# Autodesk Inventor assembly: Roller
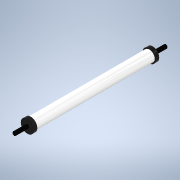
[picture p0: Inventor's stored thumbnail of the model, 180x180]
Saved by Autodesk Inventor 2020 (Build 240168000, 168)
## iProperties
Created: 2020-01-26
Part Number: Roller
Document SubType Name: Assembly
Designer: autum
Author: autum
## Documents named in this file (4)
- C:\Users\autum\Google Drive\Iron Riders 4180 (Roosevelt Robotics)\2019-2020\Build_Design\Robot 2020 (new)\Intake 2.0\Roller.iam
- C:\Users\autum\Google Drive\Iron Riders 4180 (Roosevelt Robotics)\2019-2020\Build_Design\Robot 2020 (new)\Intake 2.0\PVC Roller.ipt
- C:\Users\autum\Google Drive\Iron Riders 4180 (Roosevelt Robotics)\2019-2020\Build_Design\Robot 2020 (new)\Intake 2.0\Hex Adapter.ipt
- C:\Users\autum\Google Drive\Iron Riders 4180 (Roosevelt Robotics)\2019-2020\Build_Design\Robot 2020 (new)\Intake 2.0\Hex Instert.ipt
## Components (5 placed, 3 different names)
1. PVC Roller:1 — Insert:1, Insert:2
2. Hex Adapter:1 — Insert:1, Mate:3, Flush:2, Mate:4
3. Hex Adapter:2 — Insert:2, Mate:1, Mate:2, Flush:1
4. Hex Instert:1 — Mate:3, Flush:2, Mate:4
5. Hex Instert:2 — Mate:1, Mate:2, Flush:1
## Relationships (8: Mate 4, Insert 2, Flush 2)
- Insert:1: PVC Roller:1 ↔ Hex Adapter:1
- Insert:2: PVC Roller:1 ↔ Hex Adapter:2
- Mate:1: Hex Adapter:2 ↔ Hex Instert:2
- Mate:2: Hex Adapter:2 ↔ Hex Instert:2
- Flush:1: Hex Adapter:2 ↔ Hex Instert:2
- Mate:3: Hex Adapter:1 ↔ Hex Instert:1
- Flush:2: Hex Adapter:1 ↔ Hex Instert:1
- Mate:4: Hex Adapter:1 ↔ Hex Instert:1
